# Autodesk Inventor assembly: Lamello Bisquit Joint
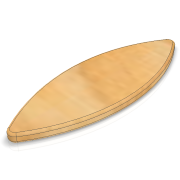
[picture p0: Inventor's stored thumbnail of the model, 180x180]
Saved by Autodesk Inventor 2024 (Build 280153000, 153)
## iProperties
RuleStatus: InUse
Created: 2022-12-20
Part Number: Lamello Bisquit Joint
Document SubType Name: Assembly
Designer: sauliusd
Author: sauliusd
## Documents named in this file (4)
- C:\W4INV 2024 Design\SMART HARDWARE\Lamello Bisquit\Lamello Bisquit Joint.iam
- C:\W4INV 2024 Design\SMART HARDWARE\Lamello Bisquit\Parts\Lamello Bisquit skeleton.ipt
- C:\W4INV 2022 Design\LIBRARY\Fixed joints\Lamello Bisquit\Lamello biscuit V2.ipt
- C:\W4INV 2024 Design\_LIBRARY\Fixed joints\Lamello Bisquit\Lamello biscuit V2\Lamello Biscuit 20.ipt
## Components (3 placed, 3 different names)
1. @Skeleton — Mate:2, Angle:1
2. Bisquit — Mate:1, Mate:2
3. Lamello Biscuit 20:2
## Component patterns: (2 elements, first: Bisquit)
## Relationships (3: Mate 2, Angle 1)
- Mate:1: Bisquit
- Angle:1 (0 deg): @Skeleton
- Mate:2: @Skeleton ↔ Bisquit
## Named parameters: ContactPatchLength = 300 mm, ContactPatchHeight = 20 mm, ConnectionAngle = 90 deg, NestledBoardT = 18 mm, PillarBoardT = 18 mm, MaxDistanceBetween = 500 mm, MinDistFromSide = 40 mm, SideDist1 = 60 mm, SideDist2 = 60 mm, MaxDistFromSide = 200 mm, Gap = 0 mm, ShiftInYDirection = 0 mm
